# Autodesk Inventor assembly: LampenkopfOhneGewinde_v1
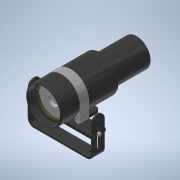
[picture p0: Inventor's stored thumbnail of the model, 180x180]
Saved by Autodesk Inventor 2020.2 (Build 242310000, 310)
## iProperties
Created: 2014-03-25
Part Number: LampenkopfOhneGewinde_v1
Document SubType Name: Assembly
Designer: schardt
Author: schardt
## Documents named in this file (16)
- C:\Users\g.schardt\Inventor\Tauchlampe\Lampenkopf.iam
- C:\Users\g.schardt\Inventor\Tauchlampe\Haltegriff.ipt
- C:\Users\g.schardt\Inventor\Tauchlampe\Glasscheibe.ipt
- C:\Users\g.schardt\Inventor\Tauchlampe\Überwurfmutter.ipt
- C:\Users\g.schardt\Inventor\Tauchlampe\Halteblech.ipt
- C:\Users\g.schardt\Inventor\Tauchlampe\Grundplattee.ipt
- C:\Users\g.schardt\Inventor\Tauchlampe\Lampengehäuse.ipt
- C:\Users\g.schardt\Inventor\Tauchlampe\Ledaufnahme.ipt
- C:\Users\g.schardt\Inventor\Tauchlampe\akkufach.iam
- C:\Users\g.schardt\Inventor\Tauchlampe\buck_3a_v4_2.ipt
- C:\Users\g.schardt\Inventor\Tauchlampe\Langmutter.IPT
- C:\Users\g.schardt\Inventor\Tauchlampe\gaggione\LLH09SPB00.ipt
- C:\Users\g.schardt\Documents\Inventor\Content Center Files\R2020\de-DE\BS 4168(8)\BS 4168 - M4 x 16(7).ipt
- C:\Users\g.schardt\Documents\Inventor\Content Center Files\R2020\de-DE\DIN 125-1  A\DIN 125 - A 3,2.ipt
- C:\Users\g.schardt\Documents\Inventor\Content Center Files\R2020\de-DE\ISO 1207(1)\DIN EN ISO 1207 - M3 x 4.ipt
- C:\Users\g.schardt\Inventor\Tauchlampe\gaggione\LLC49NMWE_mechanics_only.ipt
## Components (19 placed, 15 different names)
1. Grundplattee:1 — Passend:1, Passend:2, Fluchtend:1, Tangential:2, Fluchtend:2, Tangential:3, Passend:11, Passend:12, Passend:13, Passend:17, Passend:20, Passend:22, Passend:27, Passend:28, Passend:29, Passend:31, Passend:33, Passend:35
2. Lampengehäuse:1 — Fluchtend:1, Passend:3, Tangential:2, Tangential:3, Passend:4, Passend:5, Passend:6, Passend:7, Passend:8, Passend:9, Passend:10, Passend:14, Passend:15, Passend:16, Passend:24, Passend:37
3. Glasscheibe:1 — Passend:3, Passend:4
4. Ledaufnahme:1 — Passend:5, Passend:6, Passend:18, Passend:19, Passend:25, Passend:26, Passend:38
5. akkufach:1 [sub-assembly] — Passend:7, Passend:8
6. Überwurfmutter:1 — Passend:9, Passend:10
7. Haltegriff:1 — Passend:11, Passend:12, Passend:13, Passend:30, Passend:32
8. Halteblech:1 — Passend:14, Passend:15, Passend:17, Passend:21, Passend:23
9. buck_3a_v4_2:1 — Passend:16, Passend:18, Passend:19
10. Langmutter:1 — Passend:22, Passend:23
11. Langmutter:2 — Passend:20, Passend:21
12. LLH09SPB00:1 — Passend:24, Passend:25, Passend:26
13. BS 4168 : Teil 8 Senkkopf- und Halbrundschrauben mit Innensechskant - metrische Ausführung - Metrisch M4 x 16:1 — Passend:27
14. BS 4168 : Teil 8 Senkkopf- und Halbrundschrauben mit Innensechskant - metrische Ausführung - Metrisch M4 x 16:2 — Passend:28
15. DIN 125-1 A A 3,2:1 — Passend:29, Passend:30, Passend:36
16. DIN 125-1 A A 3,2:2 — Passend:31, Passend:32, Passend:34
17. DIN EN ISO 1207 M3 x 4:1 — Passend:33, Passend:34
18. DIN EN ISO 1207 M3 x 4:2 — Passend:35, Passend:36
19. LLC49NMWE_mechanics_only:1 — Passend:37, Passend:38
## Relationships (42: Mate 38, Flush 2, Tangent 2)
- Passend:1 [Mate]: Grundplattee:1
- Passend:2 [Mate]: Grundplattee:1
- Fluchtend:1 [Flush] (20 mm): Grundplattee:1 ↔ Lampengehäuse:1
- Passend:3 [Mate]: Lampengehäuse:1 ↔ Glasscheibe:1
- Tangential:2: Grundplattee:1 ↔ Lampengehäuse:1
- Fluchtend:2 [Flush] (-51 mm): Grundplattee:1
- Tangential:3: Grundplattee:1 ↔ Lampengehäuse:1
- Passend:4 [Mate]: Lampengehäuse:1 ↔ Glasscheibe:1
- Passend:5 [Mate]: Lampengehäuse:1 ↔ Ledaufnahme:1
- Passend:6 [Mate]: Lampengehäuse:1 ↔ Ledaufnahme:1
- Passend:7 [Mate]: Lampengehäuse:1 ↔ akkufach:1
- Passend:8 [Mate]: Lampengehäuse:1 ↔ akkufach:1
- Passend:9 [Mate]: Lampengehäuse:1 ↔ Überwurfmutter:1
- Passend:10 [Mate] (0.5 mm): Lampengehäuse:1 ↔ Überwurfmutter:1
- Passend:11 [Mate]: Grundplattee:1 ↔ Haltegriff:1
- Passend:12 [Mate]: Grundplattee:1 ↔ Haltegriff:1
- Passend:13 [Mate] (30 mm): Grundplattee:1 ↔ Haltegriff:1
- Passend:14 [Mate]: Lampengehäuse:1 ↔ Halteblech:1
- Passend:15 [Mate] (0.5 mm): Lampengehäuse:1 ↔ Halteblech:1
- Passend:16 [Mate]: Lampengehäuse:1 ↔ buck_3a_v4_2:1
- Passend:17 [Mate]: Grundplattee:1 ↔ Halteblech:1
- Passend:18 [Mate]: Ledaufnahme:1 ↔ buck_3a_v4_2:1
- Passend:19 [Mate]: Ledaufnahme:1 ↔ buck_3a_v4_2:1
- Passend:20 [Mate]: Grundplattee:1 ↔ Langmutter:2
- Passend:21 [Mate]: Halteblech:1 ↔ Langmutter:2
- Passend:22 [Mate]: Grundplattee:1 ↔ Langmutter:1
- Passend:23 [Mate]: Halteblech:1 ↔ Langmutter:1
- Passend:24 [Mate]: Lampengehäuse:1 ↔ LLH09SPB00:1
- Passend:25 [Mate]: Ledaufnahme:1 ↔ LLH09SPB00:1
- Passend:26 [Mate]: Ledaufnahme:1 ↔ LLH09SPB00:1
- Passend:27 [Mate]: Grundplattee:1 ↔ BS 4168 : Teil 8 Senkkopf- und Halbrundschrauben mit Innensechskant - metrische Ausführung - Metrisch M4 x 16:1
- Passend:28 [Mate]: Grundplattee:1 ↔ BS 4168 : Teil 8 Senkkopf- und Halbrundschrauben mit Innensechskant - metrische Ausführung - Metrisch M4 x 16:2
- Passend:29 [Mate]: Grundplattee:1 ↔ DIN 125-1 A A 3,2:1
- Passend:30 [Mate]: Haltegriff:1 ↔ DIN 125-1 A A 3,2:1
- Passend:31 [Mate]: Grundplattee:1 ↔ DIN 125-1 A A 3,2:2
- Passend:32 [Mate]: Haltegriff:1 ↔ DIN 125-1 A A 3,2:2
- Passend:33 [Mate]: Grundplattee:1 ↔ DIN EN ISO 1207 M3 x 4:1
- Passend:34 [Mate]: DIN 125-1 A A 3,2:2 ↔ DIN EN ISO 1207 M3 x 4:1
- Passend:35 [Mate]: Grundplattee:1 ↔ DIN EN ISO 1207 M3 x 4:2
- Passend:36 [Mate]: DIN 125-1 A A 3,2:1 ↔ DIN EN ISO 1207 M3 x 4:2
- Passend:37 [Mate]: Lampengehäuse:1 ↔ LLC49NMWE_mechanics_only:1
- Passend:38 [Mate]: Ledaufnahme:1 ↔ LLC49NMWE_mechanics_only:1
